# Autodesk Inventor assembly: Frame
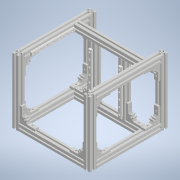
[picture p0: Inventor's stored thumbnail of the model, 180x180]
Saved by Autodesk Inventor 2022 (Build 260153000, 153)
## iProperties
Created: 2021-11-24
Part Number: Frame
Document SubType Name: Assembly
Designer: yuto6
Author: yuto6
## Documents named in this file (5)
- C:\Users\yuto6\Documents\My3DPrinter\CAD\Asm\Frame.iam
- C:\Users\yuto6\Documents\My3DPrinter\CAD\Parts\HFS3-1515-150.ipt
- C:\Users\yuto6\Documents\My3DPrinter\CAD\Parts\HFS3-1515-120.ipt
- C:\Users\yuto6\Documents\My3DPrinter\CAD\Parts\MGN7H-rail-100.iam
- C:\Users\yuto6\Documents\My3DPrinter\CAD\Parts\HBLTBS3.ipt
## Components (29 placed, 4 different names)
1. HFS3-1515-150:1 — メイト:1, メイト:3, フラッシュ:5, フラッシュ:6, フラッシュ:7, フラッシュ:8, フラッシュ:14, フラッシュ:15, メイト:26, フラッシュ:42, メイト:32, メイト:43, フラッシュ:50
2. HFS3-1515-150:2 — メイト:2, メイト:8, フラッシュ:1, フラッシュ:2, フラッシュ:3, フラッシュ:4, フラッシュ:12, フラッシュ:13, メイト:24, フラッシュ:41, メイト:30, フラッシュ:44, メイト:40
3. HFS3-1515-150:3 — メイト:7, メイト:10, メイト:22, フラッシュ:40, メイト:38
4. HFS3-1515-150:4 — メイト:4, フラッシュ:9, フラッシュ:10, メイト:11, フラッシュ:30, メイト:28, フラッシュ:43, メイト:44
5. HFS3-1515-150:5 — メイト:1, メイト:2, フラッシュ:3, フラッシュ:4, フラッシュ:5, フラッシュ:8, メイト:31, メイト:33, フラッシュ:45
6. HFS3-1515-150:7 — メイト:7, メイト:8, フラッシュ:1, フラッシュ:2, メイト:9, フラッシュ:11, メイト:23, メイト:25
7. HFS3-1515-150:8 — メイト:3, メイト:4, フラッシュ:6, フラッシュ:7, フラッシュ:9, フラッシュ:10, メイト:27, メイト:29
8. HFS3-1515-150:9 — メイト:9, フラッシュ:11, フラッシュ:17, メイト:15, メイト:16, メイト:35, フラッシュ:46, フラッシュ:47, メイト:37
9. HFS3-1515-150:10 — フラッシュ:14, フラッシュ:15, メイト:11, フラッシュ:16, メイト:18, メイト:20, フラッシュ:35, メイト:42, メイト:45, フラッシュ:51
10. HFS3-1515-150:11 — フラッシュ:12, フラッシュ:13, メイト:10, メイト:12, メイト:19, メイト:39, フラッシュ:48, メイト:41, フラッシュ:49
11. HFS3-1515-150:12 — フラッシュ:16, メイト:12, フラッシュ:17, フラッシュ:30, フラッシュ:31, フラッシュ:32
12. HFS3-1515-120:1 — フラッシュ:32, メイト:15, メイト:17, メイト:18, メイト:21, フラッシュ:38, メイト:36
13. HFS3-1515-120:2 — フラッシュ:31, メイト:16, メイト:17, フラッシュ:39, メイト:34
14. MGN7H-rail-100:1 [sub-assembly] — メイト:20, フラッシュ:33, フラッシュ:34, フラッシュ:35
15. MGN7H-rail-100:2 [sub-assembly] — メイト:19, フラッシュ:33, フラッシュ:34
16. MGN7H-rail-100:3 [sub-assembly] — フラッシュ:36, メイト:21, フラッシュ:37, フラッシュ:38
17. MGN7H-rail-100:4 [sub-assembly] — フラッシュ:36, フラッシュ:37, フラッシュ:39
18. HBLTBS3:1 — メイト:28, メイト:29, フラッシュ:43
19. HBLTBS3:2 — メイト:22, メイト:23, フラッシュ:40
20. HBLTBS3:3 — メイト:24, メイト:25, フラッシュ:41
21. HBLTBS3:4 — メイト:26, メイト:27, フラッシュ:42
22. HBLTBS3:5 — メイト:30, メイト:31, フラッシュ:44
23. HBLTBS3:6 — メイト:32, メイト:33, フラッシュ:45
24. HBLTBS3:7 — メイト:34, メイト:35, フラッシュ:46
25. HBLTBS3:8 — フラッシュ:47, メイト:36, メイト:37
26. HBLTBS3:9 — メイト:38, メイト:39, フラッシュ:48
27. HBLTBS3:10 — メイト:44, メイト:45, フラッシュ:51
28. HBLTBS3:11 — メイト:40, メイト:41, フラッシュ:49
29. HBLTBS3:12 — メイト:42, メイト:43, フラッシュ:50
## Relationships (80: Mate 41, Flush 39)
- メイト:1 [Mate]: HFS3-1515-150:1 ↔ HFS3-1515-150:5
- メイト:2 [Mate]: HFS3-1515-150:2 ↔ HFS3-1515-150:5
- メイト:3 [Mate]: HFS3-1515-150:1 ↔ HFS3-1515-150:8
- メイト:4 [Mate]: HFS3-1515-150:4 ↔ HFS3-1515-150:8
- メイト:7 [Mate]: HFS3-1515-150:3 ↔ HFS3-1515-150:7
- メイト:8 [Mate]: HFS3-1515-150:2 ↔ HFS3-1515-150:7
- フラッシュ:1 [Flush]: HFS3-1515-150:2 ↔ HFS3-1515-150:7
- フラッシュ:2 [Flush]: HFS3-1515-150:2 ↔ HFS3-1515-150:7
- フラッシュ:3 [Flush]: HFS3-1515-150:2 ↔ HFS3-1515-150:5
- フラッシュ:4 [Flush]: HFS3-1515-150:2 ↔ HFS3-1515-150:5
- フラッシュ:5 [Flush]: HFS3-1515-150:1 ↔ HFS3-1515-150:5
- フラッシュ:6 [Flush]: HFS3-1515-150:1 ↔ HFS3-1515-150:8
- フラッシュ:7 [Flush]: HFS3-1515-150:1 ↔ HFS3-1515-150:8
- フラッシュ:8 [Flush]: HFS3-1515-150:1 ↔ HFS3-1515-150:5
- フラッシュ:9 [Flush]: HFS3-1515-150:4 ↔ HFS3-1515-150:8
- フラッシュ:10 [Flush]: HFS3-1515-150:4 ↔ HFS3-1515-150:8
- メイト:9 [Mate]: HFS3-1515-150:7 ↔ HFS3-1515-150:9
- フラッシュ:11 [Flush]: HFS3-1515-150:7 ↔ HFS3-1515-150:9
- フラッシュ:12 [Flush]: HFS3-1515-150:2 ↔ HFS3-1515-150:11
- フラッシュ:13 [Flush]: HFS3-1515-150:2 ↔ HFS3-1515-150:11
- メイト:10 [Mate]: HFS3-1515-150:3 ↔ HFS3-1515-150:11
- フラッシュ:14 [Flush]: HFS3-1515-150:1 ↔ HFS3-1515-150:10
- フラッシュ:15 [Flush]: HFS3-1515-150:1 ↔ HFS3-1515-150:10
- メイト:11 [Mate]: HFS3-1515-150:4 ↔ HFS3-1515-150:10
- フラッシュ:16 [Flush]: HFS3-1515-150:10 ↔ HFS3-1515-150:12
- メイト:12 [Mate]: HFS3-1515-150:11 ↔ HFS3-1515-150:12
- フラッシュ:17 [Flush]: HFS3-1515-150:9 ↔ HFS3-1515-150:12
- フラッシュ:30 [Flush] (37 mm): HFS3-1515-150:4 ↔ HFS3-1515-150:12
- フラッシュ:31 [Flush]: HFS3-1515-150:12 ↔ HFS3-1515-120:2
- フラッシュ:32 [Flush]: HFS3-1515-150:12 ↔ HFS3-1515-120:1
- メイト:15 [Mate]: HFS3-1515-150:9 ↔ HFS3-1515-120:1
- メイト:16 [Mate]: HFS3-1515-150:9 ↔ HFS3-1515-120:2
- メイト:17 [Mate] (54 mm): HFS3-1515-120:1 ↔ HFS3-1515-120:2
- メイト:18 [Mate] (33 mm): HFS3-1515-150:10 ↔ HFS3-1515-120:1
- メイト:19 [Mate]: HFS3-1515-150:11 ↔ MGN7H-rail-100:2
- メイト:20 [Mate]: HFS3-1515-150:10 ↔ MGN7H-rail-100:1
- フラッシュ:33 [Flush]: MGN7H-rail-100:1 ↔ MGN7H-rail-100:2
- フラッシュ:34 [Flush]: MGN7H-rail-100:1 ↔ MGN7H-rail-100:2
- フラッシュ:35 [Flush] (4 mm): HFS3-1515-150:10 ↔ MGN7H-rail-100:1
- フラッシュ:36 [Flush]: MGN7H-rail-100:3 ↔ MGN7H-rail-100:4
- メイト:21 [Mate]: HFS3-1515-120:1 ↔ MGN7H-rail-100:3
- フラッシュ:37 [Flush]: MGN7H-rail-100:3 ↔ MGN7H-rail-100:4
- フラッシュ:38 [Flush] (4 mm): HFS3-1515-120:1 ↔ MGN7H-rail-100:3
- フラッシュ:39 [Flush] (4 mm): HFS3-1515-120:2 ↔ MGN7H-rail-100:4
- メイト:22 [Mate]: HFS3-1515-150:3 ↔ HBLTBS3:2
- メイト:23 [Mate]: HFS3-1515-150:7 ↔ HBLTBS3:2
- フラッシュ:40 [Flush] (3 mm): HFS3-1515-150:3 ↔ HBLTBS3:2
- メイト:24 [Mate]: HFS3-1515-150:2 ↔ HBLTBS3:3
- メイト:25 [Mate]: HFS3-1515-150:7 ↔ HBLTBS3:3
- フラッシュ:41 [Flush] (3 mm): HFS3-1515-150:2 ↔ HBLTBS3:3
- メイト:26 [Mate]: HFS3-1515-150:1 ↔ HBLTBS3:4
- メイト:27 [Mate]: HFS3-1515-150:8 ↔ HBLTBS3:4
- フラッシュ:42 [Flush] (3 mm): HFS3-1515-150:1 ↔ HBLTBS3:4
- メイト:28 [Mate]: HFS3-1515-150:4 ↔ HBLTBS3:1
- メイト:29 [Mate]: HFS3-1515-150:8 ↔ HBLTBS3:1
- フラッシュ:43 [Flush] (3 mm): HFS3-1515-150:4 ↔ HBLTBS3:1
- メイト:30 [Mate]: HFS3-1515-150:2 ↔ HBLTBS3:5
- メイト:31 [Mate]: HFS3-1515-150:5 ↔ HBLTBS3:5
- フラッシュ:44 [Flush] (3 mm): HFS3-1515-150:2 ↔ HBLTBS3:5
- メイト:32 [Mate]: HFS3-1515-150:1 ↔ HBLTBS3:6
- メイト:33 [Mate]: HFS3-1515-150:5 ↔ HBLTBS3:6
- フラッシュ:45 [Flush] (3 mm): HFS3-1515-150:5 ↔ HBLTBS3:6
- メイト:34 [Mate]: HFS3-1515-120:2 ↔ HBLTBS3:7
- メイト:35 [Mate]: HFS3-1515-150:9 ↔ HBLTBS3:7
- フラッシュ:46 [Flush] (3 mm): HFS3-1515-150:9 ↔ HBLTBS3:7
- フラッシュ:47 [Flush] (3 mm): HFS3-1515-150:9 ↔ HBLTBS3:8
- メイト:36 [Mate]: HFS3-1515-120:1 ↔ HBLTBS3:8
- メイト:37 [Mate]: HFS3-1515-150:9 ↔ HBLTBS3:8
- メイト:38 [Mate]: HFS3-1515-150:3 ↔ HBLTBS3:9
- メイト:39 [Mate]: HFS3-1515-150:11 ↔ HBLTBS3:9
- フラッシュ:48 [Flush] (3 mm): HFS3-1515-150:11 ↔ HBLTBS3:9
- メイト:40 [Mate]: HFS3-1515-150:2 ↔ HBLTBS3:11
- メイト:41 [Mate]: HFS3-1515-150:11 ↔ HBLTBS3:11
- フラッシュ:49 [Flush] (3 mm): HFS3-1515-150:11 ↔ HBLTBS3:11
- メイト:42 [Mate]: HFS3-1515-150:10 ↔ HBLTBS3:12
- メイト:43 [Mate]: HFS3-1515-150:1 ↔ HBLTBS3:12
- フラッシュ:50 [Flush] (3 mm): HFS3-1515-150:1 ↔ HBLTBS3:12
- メイト:44 [Mate]: HFS3-1515-150:4 ↔ HBLTBS3:10
- メイト:45 [Mate]: HFS3-1515-150:10 ↔ HBLTBS3:10
- フラッシュ:51 [Flush] (3 mm): HFS3-1515-150:10 ↔ HBLTBS3:10
